# Autodesk Inventor assembly: SPE0V1 Ensamble General
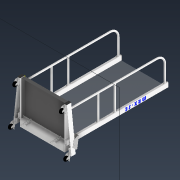
[picture p0: Inventor's stored thumbnail of the model, 180x180]
Saved by Autodesk Inventor 2021.2 (Build 252289000, 289)
## iProperties
Created: 2026-05-12
Part Number: SPE0V1 Ensamble General
Document SubType Name: Assembly
Designer: nelso
Author: nelso
## Documents named in this file (11)
- C:\Users\Tecnica\OneDrive\Documentos\Mecanica\Soporte-Paciente-Espinografia\Workspace\SPE0V1 Ensamble General.iam
- C:\Users\Tecnica\OneDrive\Documentos\Mecanica\Soporte-Paciente-Espinografia\Workspace\SP25V1 Acrilico.ipt
- C:\Users\Tecnica\OneDrive\Documentos\Mecanica\Soporte-Paciente-Espinografia\Workspace\SPE1V1 Estructura.iam
- C:\Users\Tecnica\OneDrive\Documentos\Mecanica\Soporte-Paciente-Espinografia\Workspace\SPE2V1 Baranda.iam
- C:\Users\Tecnica\OneDrive\Documentos\Mecanica\Soporte-Paciente-Espinografia\Workspace\DIN933M8X1.25L20C.ipt
- C:\Users\Tecnica\OneDrive\Documentos\Mecanica\Soporte-Paciente-Espinografia\Workspace\DIN125-A8,4C.ipt
- C:\Users\Tecnica\OneDrive\Documentos\Mecanica\Soporte-Paciente-Espinografia\Workspace\Logo.ipt
- C:\Users\Tecnica\OneDrive\Documentos\Mecanica\Soporte-Paciente-Espinografia\Workspace\SP16V1 Seguro Acrilico.ipt
- C:\Users\Tecnica\OneDrive\Documentos\Mecanica\Soporte-Paciente-Espinografia\Workspace\RFPLUS4PO300 Tuerca rem M4 cab red.ipt
- C:\Users\Tecnica\OneDrive\Documentos\Mecanica\Soporte-Paciente-Espinografia\Workspace\ISO7380M4X0.8L12I.ipt
- C:\Users\Tecnica\OneDrive\Documentos\Mecanica\Soporte-Paciente-Espinografia\Workspace\SP26V1 Base Chapa.ipt
## Components (76 placed, 10 different names)
1. SP26V1 Base Chapa:1 — Flush:17, Mate:178, Mate:242
2. SP25V1 Acrilico:1 — Mate:71, Mate:179, Mate:180, Flush:19, Flush:20, Mate:261, Mate:262
3. SPE1V1 Estructura:1 [sub-assembly] — Mate:71, Coincidencia:100, Coincidencia:101, Coincidencia:102, Coincidencia:117, Nivelación:14, Nivelación:15, Flush:17, Mate:178, Flush:23, Flush:24, Flush:25, Flush:26, Flush:27, Flush:28, Flush:29, Flush:30, Flush:31, Mate:235, Mate:236, Mate:237, Flush:32, Flush:33, Flush:34, Flush:35, Flush:36, Flush:37, Flush:38, Flush:39, Flush:40, Mate:239, Mate:240, Mate:241, Mate:242, Flush:41, Flush:42, Mate:243, Mate:244, Mate:245, Mate:246, Mate:247, Mate:248, Mate:249, Mate:250, Mate:251, Mate:252, Mate:253, Mate:254, Mate:255, Mate:256, Mate:257, Mate:258, Mate:259, Mate:260
4. SPE2V1 Baranda:2 [sub-assembly] — Coincidencia:100, Coincidencia:101, Coincidencia:102, Coincidencia:109, Coincidencia:110, Coincidencia:111, Coincidencia:112, Mate:134, Mate:135, Mate:136, Mate:137, Mate:138, Mate:139, Mate:140, Mate:141, Mate:142, Mate:143, Mate:144, Mate:145, Mate:168, Mate:169, Mate:170, Mate:171, Mate:172, Mate:173
5. SPE2V1 Baranda:3 [sub-assembly] — Mate:118, Mate:119, Mate:120, Mate:121, Mate:122, Mate:123, Mate:124, Mate:125, Mate:126, Mate:127, Mate:128, Mate:129, Mate:130, Mate:131, Mate:132, Mate:133, Mate:147, Mate:149, Mate:156, Mate:157, Mate:158, Mate:159, Mate:160, Mate:161, Mate:235, Mate:236
6. DIN933M8X1.25L20C:1 — Coincidencia:113, Coincidencia:114
7. DIN125-A8,4C:1 — Coincidencia:109, Coincidencia:110, Coincidencia:115, Coincidencia:116
8. DIN125-A8,4C:2 — Coincidencia:111, Coincidencia:112, Coincidencia:113, Coincidencia:114
9. DIN933M8X1.25L20C:2 — Coincidencia:115, Coincidencia:116
10. Logo:1 — Coincidencia:117, Nivelación:14, Nivelación:15
11. DIN125-A8,4C:3 — Mate:144, Mate:145, Mate:162
12. DIN125-A8,4C:4 — Mate:142, Mate:143, Mate:163
13. DIN125-A8,4C:5 — Mate:140, Mate:141, Mate:164
14. DIN125-A8,4C:6 — Mate:138, Mate:139, Mate:165
15. DIN125-A8,4C:7 — Mate:135, Mate:136, Mate:167
16. DIN125-A8,4C:8 — Mate:134, Mate:137, Mate:166
17. DIN125-A8,4C:9 — Mate:130, Mate:132, Mate:155
18. DIN125-A8,4C:10 — Mate:131, Mate:133, Mate:154
19. DIN125-A8,4C:11 — Mate:128, Mate:129, Mate:153
20. DIN125-A8,4C:12 — Mate:126, Mate:127, Mate:152
21. DIN125-A8,4C:13 — Mate:122, Mate:123, Mate:150
22. DIN125-A8,4C:14 — Mate:124, Mate:125, Mate:151
23. DIN125-A8,4C:15 — Mate:120, Mate:121, Mate:148
24. DIN125-A8,4C:16 — Mate:118, Mate:119, Mate:146
25. DIN933M8X1.25L20C:3 — Mate:162, Mate:168
26. DIN933M8X1.25L20C:4 — Mate:163, Mate:169
27. DIN933M8X1.25L20C:5 — Mate:164, Mate:170
28. DIN933M8X1.25L20C:6 — Mate:165, Mate:171
29. DIN933M8X1.25L20C:7 — Mate:166, Mate:172
30. DIN933M8X1.25L20C:8 — Mate:167, Mate:173
31. DIN933M8X1.25L20C:9 — Mate:155, Mate:156
32. DIN933M8X1.25L20C:10 — Mate:154, Mate:157
33. DIN933M8X1.25L20C:11 — Mate:153, Mate:159
34. DIN933M8X1.25L20C:12 — Mate:152, Mate:158
35. DIN933M8X1.25L20C:13 — Mate:151, Mate:160
36. DIN933M8X1.25L20C:14 — Mate:150, Mate:161, Mate:237
37. DIN933M8X1.25L20C:15 — Mate:148, Mate:149
38. DIN933M8X1.25L20C:16 — Mate:146, Mate:147
39. SP16V1 Seguro Acrilico:1 — Mate:179, Flush:19, Mate:181, Mate:199, Mate:200, Mate:201, Mate:202, Mate:203, Mate:204, Mate:205, Mate:206, Mate:207, Mate:217, Mate:218, Mate:219, Mate:220, Mate:221, Mate:222, Mate:223, Mate:224, Mate:225
40. SP16V1 Seguro Acrilico:2 — Mate:180, Flush:20, Mate:208, Mate:209, Mate:210, Mate:211, Mate:212, Mate:213, Mate:214, Mate:215, Mate:216, Mate:226, Mate:227, Mate:228, Mate:229, Mate:230, Mate:231, Mate:232, Mate:233, Mate:234, Flush:40, Flush:42
41. RFPLUS4PO300 Tuerca rem M4 cab red:1 — Mate:181, Flush:23, Mate:251
42. RFPLUS4PO300 Tuerca rem M4 cab red:2 — Flush:24, Mate:250
43. RFPLUS4PO300 Tuerca rem M4 cab red:3 — Flush:25, Mate:249
44. RFPLUS4PO300 Tuerca rem M4 cab red:4 — Flush:26, Mate:248
45. RFPLUS4PO300 Tuerca rem M4 cab red:5 — Flush:27, Mate:247
46. RFPLUS4PO300 Tuerca rem M4 cab red:6 — Flush:28, Mate:246
47. RFPLUS4PO300 Tuerca rem M4 cab red:7 — Flush:29, Mate:245
48. RFPLUS4PO300 Tuerca rem M4 cab red:8 — Flush:30, Mate:244
49. RFPLUS4PO300 Tuerca rem M4 cab red:9 — Flush:31, Mate:243
50. RFPLUS4PO300 Tuerca rem M4 cab red:10 — Flush:32, Mate:252, Mate:261
51. RFPLUS4PO300 Tuerca rem M4 cab red:11 — Flush:33, Mate:253
52. RFPLUS4PO300 Tuerca rem M4 cab red:12 — Flush:34, Mate:254
53. RFPLUS4PO300 Tuerca rem M4 cab red:13 — Flush:35, Mate:255
54. RFPLUS4PO300 Tuerca rem M4 cab red:14 — Flush:36, Mate:256
55. RFPLUS4PO300 Tuerca rem M4 cab red:15 — Flush:37, Mate:257
56. RFPLUS4PO300 Tuerca rem M4 cab red:16 — Flush:38, Mate:258
57. RFPLUS4PO300 Tuerca rem M4 cab red:17 — Flush:39, Mate:259
58. RFPLUS4PO300 Tuerca rem M4 cab red:18 — Flush:41, Mate:260
59. ISO7380M4X0.8L12I:1 — Mate:199, Mate:217
60. ISO7380M4X0.8L12I:2 — Mate:200, Mate:218
61. ISO7380M4X0.8L12I:3 — Mate:201, Mate:219
62. ISO7380M4X0.8L12I:4 — Mate:202, Mate:220
63. ISO7380M4X0.8L12I:5 — Mate:203, Mate:221
64. ISO7380M4X0.8L12I:6 — Mate:204, Mate:222
65. ISO7380M4X0.8L12I:7 — Mate:205, Mate:223
66. ISO7380M4X0.8L12I:8 — Mate:206, Mate:224
67. ISO7380M4X0.8L12I:9 — Mate:207, Mate:225
68. ISO7380M4X0.8L12I:10 — Mate:208, Mate:234, Mate:262
69. ISO7380M4X0.8L12I:11 — Mate:209, Mate:233
70. ISO7380M4X0.8L12I:12 — Mate:210, Mate:232
71. ISO7380M4X0.8L12I:13 — Mate:211, Mate:231
72. ISO7380M4X0.8L12I:14 — Mate:212, Mate:230
73. ISO7380M4X0.8L12I:15 — Mate:214, Mate:228
74. ISO7380M4X0.8L12I:16 — Mate:215, Mate:227
75. ISO7380M4X0.8L12I:17 — Mate:216, Mate:226
76. ISO7380M4X0.8L12I:18 — Mate:213, Mate:229
## Relationships (161: Mate 136, Flush 25)
- Mate:71: SP25V1 Acrilico:1 ↔ SPE1V1 Estructura:1
- Coincidencia:100 [Mate]: SPE1V1 Estructura:1 ↔ SPE2V1 Baranda:2
- Coincidencia:101 [Mate]: SPE1V1 Estructura:1 ↔ SPE2V1 Baranda:2
- Coincidencia:102 [Mate]: SPE1V1 Estructura:1 ↔ SPE2V1 Baranda:2
- Coincidencia:109 [Mate]: SPE2V1 Baranda:2 ↔ DIN125-A8,4C:1
- Coincidencia:110 [Mate]: SPE2V1 Baranda:2 ↔ DIN125-A8,4C:1
- Coincidencia:111 [Mate]: SPE2V1 Baranda:2 ↔ DIN125-A8,4C:2
- Coincidencia:112 [Mate]: SPE2V1 Baranda:2 ↔ DIN125-A8,4C:2
- Coincidencia:113 [Mate]: DIN933M8X1.25L20C:1 ↔ DIN125-A8,4C:2
- Coincidencia:114 [Mate]: DIN933M8X1.25L20C:1 ↔ DIN125-A8,4C:2
- Coincidencia:115 [Mate]: DIN125-A8,4C:1 ↔ DIN933M8X1.25L20C:2
- Coincidencia:116 [Mate]: DIN125-A8,4C:1 ↔ DIN933M8X1.25L20C:2
- Coincidencia:117 [Mate]: SPE1V1 Estructura:1 ↔ Logo:1
- Nivelación:14 [Flush] (10 mm): SPE1V1 Estructura:1 ↔ Logo:1
- Nivelación:15 [Flush] (400 mm): SPE1V1 Estructura:1 ↔ Logo:1
- Mate:118: SPE2V1 Baranda:3 ↔ DIN125-A8,4C:16
- Mate:119: SPE2V1 Baranda:3 ↔ DIN125-A8,4C:16
- Mate:120: SPE2V1 Baranda:3 ↔ DIN125-A8,4C:15
- Mate:121: SPE2V1 Baranda:3 ↔ DIN125-A8,4C:15
- Mate:122: SPE2V1 Baranda:3 ↔ DIN125-A8,4C:13
- Mate:123: SPE2V1 Baranda:3 ↔ DIN125-A8,4C:13
- Mate:124: SPE2V1 Baranda:3 ↔ DIN125-A8,4C:14
- Mate:125: SPE2V1 Baranda:3 ↔ DIN125-A8,4C:14
- Mate:126: SPE2V1 Baranda:3 ↔ DIN125-A8,4C:12
- Mate:127: SPE2V1 Baranda:3 ↔ DIN125-A8,4C:12
- Mate:128: SPE2V1 Baranda:3 ↔ DIN125-A8,4C:11
- Mate:129: SPE2V1 Baranda:3 ↔ DIN125-A8,4C:11
- Mate:130: SPE2V1 Baranda:3 ↔ DIN125-A8,4C:9
- Mate:131: SPE2V1 Baranda:3 ↔ DIN125-A8,4C:10
- Mate:132: SPE2V1 Baranda:3 ↔ DIN125-A8,4C:9
- Mate:133: SPE2V1 Baranda:3 ↔ DIN125-A8,4C:10
- Mate:134: SPE2V1 Baranda:2 ↔ DIN125-A8,4C:8
- Mate:135: SPE2V1 Baranda:2 ↔ DIN125-A8,4C:7
- Mate:136: SPE2V1 Baranda:2 ↔ DIN125-A8,4C:7
- Mate:137: SPE2V1 Baranda:2 ↔ DIN125-A8,4C:8
- Mate:138: SPE2V1 Baranda:2 ↔ DIN125-A8,4C:6
- Mate:139: SPE2V1 Baranda:2 ↔ DIN125-A8,4C:6
- Mate:140: SPE2V1 Baranda:2 ↔ DIN125-A8,4C:5
- Mate:141: SPE2V1 Baranda:2 ↔ DIN125-A8,4C:5
- Mate:142: SPE2V1 Baranda:2 ↔ DIN125-A8,4C:4
- Mate:143: SPE2V1 Baranda:2 ↔ DIN125-A8,4C:4
- Mate:144: SPE2V1 Baranda:2 ↔ DIN125-A8,4C:3
- Mate:145: SPE2V1 Baranda:2 ↔ DIN125-A8,4C:3
- Mate:146: DIN125-A8,4C:16 ↔ DIN933M8X1.25L20C:16
- Mate:147: SPE2V1 Baranda:3 ↔ DIN933M8X1.25L20C:16
- Mate:148: DIN125-A8,4C:15 ↔ DIN933M8X1.25L20C:15
- Mate:149: SPE2V1 Baranda:3 ↔ DIN933M8X1.25L20C:15
- Mate:150: DIN125-A8,4C:13 ↔ DIN933M8X1.25L20C:14
- Mate:151: DIN125-A8,4C:14 ↔ DIN933M8X1.25L20C:13
- Mate:152: DIN125-A8,4C:12 ↔ DIN933M8X1.25L20C:12
- Mate:153: DIN125-A8,4C:11 ↔ DIN933M8X1.25L20C:11
- Mate:154: DIN125-A8,4C:10 ↔ DIN933M8X1.25L20C:10
- Mate:155: DIN125-A8,4C:9 ↔ DIN933M8X1.25L20C:9
- Mate:156: SPE2V1 Baranda:3 ↔ DIN933M8X1.25L20C:9
- Mate:157: SPE2V1 Baranda:3 ↔ DIN933M8X1.25L20C:10
- Mate:158: SPE2V1 Baranda:3 ↔ DIN933M8X1.25L20C:12
- Mate:159: SPE2V1 Baranda:3 ↔ DIN933M8X1.25L20C:11
- Mate:160: SPE2V1 Baranda:3 ↔ DIN933M8X1.25L20C:13
- Mate:161: SPE2V1 Baranda:3 ↔ DIN933M8X1.25L20C:14
- Mate:162: DIN125-A8,4C:3 ↔ DIN933M8X1.25L20C:3
- Mate:163: DIN125-A8,4C:4 ↔ DIN933M8X1.25L20C:4
- Mate:164: DIN125-A8,4C:5 ↔ DIN933M8X1.25L20C:5
- Mate:165: DIN125-A8,4C:6 ↔ DIN933M8X1.25L20C:6
- Mate:166: DIN125-A8,4C:8 ↔ DIN933M8X1.25L20C:7
- Mate:167: DIN125-A8,4C:7 ↔ DIN933M8X1.25L20C:8
- Mate:168: SPE2V1 Baranda:2 ↔ DIN933M8X1.25L20C:3
- Mate:169: SPE2V1 Baranda:2 ↔ DIN933M8X1.25L20C:4
- Mate:170: SPE2V1 Baranda:2 ↔ DIN933M8X1.25L20C:5
- Mate:171: SPE2V1 Baranda:2 ↔ DIN933M8X1.25L20C:6
- Mate:172: SPE2V1 Baranda:2 ↔ DIN933M8X1.25L20C:7
- Mate:173: SPE2V1 Baranda:2 ↔ DIN933M8X1.25L20C:8
- Flush:17: SP26V1 Base Chapa:1 ↔ SPE1V1 Estructura:1
- Mate:178 (5 mm): SP26V1 Base Chapa:1 ↔ SPE1V1 Estructura:1
- Mate:179: SP25V1 Acrilico:1 ↔ SP16V1 Seguro Acrilico:1
- Mate:180: SP25V1 Acrilico:1 ↔ SP16V1 Seguro Acrilico:2
- Flush:19: SP25V1 Acrilico:1 ↔ SP16V1 Seguro Acrilico:1
- Flush:20: SP25V1 Acrilico:1 ↔ SP16V1 Seguro Acrilico:2
- Mate:181: SP16V1 Seguro Acrilico:1 ↔ RFPLUS4PO300 Tuerca rem M4 cab red:1
- Flush:23: SPE1V1 Estructura:1 ↔ RFPLUS4PO300 Tuerca rem M4 cab red:1
- Flush:24: SPE1V1 Estructura:1 ↔ RFPLUS4PO300 Tuerca rem M4 cab red:2
- Flush:25: SPE1V1 Estructura:1 ↔ RFPLUS4PO300 Tuerca rem M4 cab red:3
- Flush:26: SPE1V1 Estructura:1 ↔ RFPLUS4PO300 Tuerca rem M4 cab red:4
- Flush:27: SPE1V1 Estructura:1 ↔ RFPLUS4PO300 Tuerca rem M4 cab red:5
- Flush:28: SPE1V1 Estructura:1 ↔ RFPLUS4PO300 Tuerca rem M4 cab red:6
- Flush:29: SPE1V1 Estructura:1 ↔ RFPLUS4PO300 Tuerca rem M4 cab red:7
- Flush:30: SPE1V1 Estructura:1 ↔ RFPLUS4PO300 Tuerca rem M4 cab red:8
- Flush:31: SPE1V1 Estructura:1 ↔ RFPLUS4PO300 Tuerca rem M4 cab red:9
- Mate:199: SP16V1 Seguro Acrilico:1 ↔ ISO7380M4X0.8L12I:1
- Mate:200: SP16V1 Seguro Acrilico:1 ↔ ISO7380M4X0.8L12I:2
- Mate:201: SP16V1 Seguro Acrilico:1 ↔ ISO7380M4X0.8L12I:3
- Mate:202: SP16V1 Seguro Acrilico:1 ↔ ISO7380M4X0.8L12I:4
- Mate:203: SP16V1 Seguro Acrilico:1 ↔ ISO7380M4X0.8L12I:5
- Mate:204: SP16V1 Seguro Acrilico:1 ↔ ISO7380M4X0.8L12I:6
- Mate:205: SP16V1 Seguro Acrilico:1 ↔ ISO7380M4X0.8L12I:7
- Mate:206: SP16V1 Seguro Acrilico:1 ↔ ISO7380M4X0.8L12I:8
- Mate:207: SP16V1 Seguro Acrilico:1 ↔ ISO7380M4X0.8L12I:9
- Mate:208: SP16V1 Seguro Acrilico:2 ↔ ISO7380M4X0.8L12I:10
- Mate:209: SP16V1 Seguro Acrilico:2 ↔ ISO7380M4X0.8L12I:11
- Mate:210: SP16V1 Seguro Acrilico:2 ↔ ISO7380M4X0.8L12I:12
- Mate:211: SP16V1 Seguro Acrilico:2 ↔ ISO7380M4X0.8L12I:13
- Mate:212: SP16V1 Seguro Acrilico:2 ↔ ISO7380M4X0.8L12I:14
- Mate:213: SP16V1 Seguro Acrilico:2 ↔ ISO7380M4X0.8L12I:18
- Mate:214: SP16V1 Seguro Acrilico:2 ↔ ISO7380M4X0.8L12I:15
- Mate:215: SP16V1 Seguro Acrilico:2 ↔ ISO7380M4X0.8L12I:16
- Mate:216: SP16V1 Seguro Acrilico:2 ↔ ISO7380M4X0.8L12I:17
- Mate:217: SP16V1 Seguro Acrilico:1 ↔ ISO7380M4X0.8L12I:1
- Mate:218: SP16V1 Seguro Acrilico:1 ↔ ISO7380M4X0.8L12I:2
- Mate:219: SP16V1 Seguro Acrilico:1 ↔ ISO7380M4X0.8L12I:3
- Mate:220: SP16V1 Seguro Acrilico:1 ↔ ISO7380M4X0.8L12I:4
- Mate:221: SP16V1 Seguro Acrilico:1 ↔ ISO7380M4X0.8L12I:5
- Mate:222: SP16V1 Seguro Acrilico:1 ↔ ISO7380M4X0.8L12I:6
- Mate:223: SP16V1 Seguro Acrilico:1 ↔ ISO7380M4X0.8L12I:7
- Mate:224: SP16V1 Seguro Acrilico:1 ↔ ISO7380M4X0.8L12I:8
- Mate:225: SP16V1 Seguro Acrilico:1 ↔ ISO7380M4X0.8L12I:9
- Mate:226: SP16V1 Seguro Acrilico:2 ↔ ISO7380M4X0.8L12I:17
- Mate:227: SP16V1 Seguro Acrilico:2 ↔ ISO7380M4X0.8L12I:16
- Mate:228: SP16V1 Seguro Acrilico:2 ↔ ISO7380M4X0.8L12I:15
- Mate:229: SP16V1 Seguro Acrilico:2 ↔ ISO7380M4X0.8L12I:18
- Mate:230: SP16V1 Seguro Acrilico:2 ↔ ISO7380M4X0.8L12I:14
- Mate:231: SP16V1 Seguro Acrilico:2 ↔ ISO7380M4X0.8L12I:13
- Mate:232: SP16V1 Seguro Acrilico:2 ↔ ISO7380M4X0.8L12I:12
- Mate:233: SP16V1 Seguro Acrilico:2 ↔ ISO7380M4X0.8L12I:11
- Mate:234: SP16V1 Seguro Acrilico:2 ↔ ISO7380M4X0.8L12I:10
- Mate:235: SPE1V1 Estructura:1 ↔ SPE2V1 Baranda:3
- Mate:236: SPE1V1 Estructura:1 ↔ SPE2V1 Baranda:3
- Mate:237: SPE1V1 Estructura:1 ↔ DIN933M8X1.25L20C:14
- Flush:32: SPE1V1 Estructura:1 ↔ RFPLUS4PO300 Tuerca rem M4 cab red:10
- Flush:33: SPE1V1 Estructura:1 ↔ RFPLUS4PO300 Tuerca rem M4 cab red:11
- Flush:34: SPE1V1 Estructura:1 ↔ RFPLUS4PO300 Tuerca rem M4 cab red:12
- Flush:35: SPE1V1 Estructura:1 ↔ RFPLUS4PO300 Tuerca rem M4 cab red:13
- Flush:36: SPE1V1 Estructura:1 ↔ RFPLUS4PO300 Tuerca rem M4 cab red:14
- Flush:37: SPE1V1 Estructura:1 ↔ RFPLUS4PO300 Tuerca rem M4 cab red:15
- Flush:38: SPE1V1 Estructura:1 ↔ RFPLUS4PO300 Tuerca rem M4 cab red:16
- Flush:39: SPE1V1 Estructura:1 ↔ RFPLUS4PO300 Tuerca rem M4 cab red:17
- Flush:40: SPE1V1 Estructura:1 ↔ SP16V1 Seguro Acrilico:2
- Mate:239: SPE1V1 Estructura:1
- Mate:240: SPE1V1 Estructura:1
- Mate:241: SPE1V1 Estructura:1
- Mate:242: SP26V1 Base Chapa:1 ↔ SPE1V1 Estructura:1
- Flush:41: SPE1V1 Estructura:1 ↔ RFPLUS4PO300 Tuerca rem M4 cab red:18
- Flush:42: SPE1V1 Estructura:1 ↔ SP16V1 Seguro Acrilico:2
- Mate:243: SPE1V1 Estructura:1 ↔ RFPLUS4PO300 Tuerca rem M4 cab red:9
- Mate:244: SPE1V1 Estructura:1 ↔ RFPLUS4PO300 Tuerca rem M4 cab red:8
- Mate:245: SPE1V1 Estructura:1 ↔ RFPLUS4PO300 Tuerca rem M4 cab red:7
- Mate:246: SPE1V1 Estructura:1 ↔ RFPLUS4PO300 Tuerca rem M4 cab red:6
- Mate:247: SPE1V1 Estructura:1 ↔ RFPLUS4PO300 Tuerca rem M4 cab red:5
- Mate:248: SPE1V1 Estructura:1 ↔ RFPLUS4PO300 Tuerca rem M4 cab red:4
- Mate:249: SPE1V1 Estructura:1 ↔ RFPLUS4PO300 Tuerca rem M4 cab red:3
- Mate:250: SPE1V1 Estructura:1 ↔ RFPLUS4PO300 Tuerca rem M4 cab red:2
- Mate:251: SPE1V1 Estructura:1 ↔ RFPLUS4PO300 Tuerca rem M4 cab red:1
- Mate:252: SPE1V1 Estructura:1 ↔ RFPLUS4PO300 Tuerca rem M4 cab red:10
- Mate:253: SPE1V1 Estructura:1 ↔ RFPLUS4PO300 Tuerca rem M4 cab red:11
- Mate:254: SPE1V1 Estructura:1 ↔ RFPLUS4PO300 Tuerca rem M4 cab red:12
- Mate:255: SPE1V1 Estructura:1 ↔ RFPLUS4PO300 Tuerca rem M4 cab red:13
- Mate:256: SPE1V1 Estructura:1 ↔ RFPLUS4PO300 Tuerca rem M4 cab red:14
- Mate:257: SPE1V1 Estructura:1 ↔ RFPLUS4PO300 Tuerca rem M4 cab red:15
- Mate:258: SPE1V1 Estructura:1 ↔ RFPLUS4PO300 Tuerca rem M4 cab red:16
- Mate:259: SPE1V1 Estructura:1 ↔ RFPLUS4PO300 Tuerca rem M4 cab red:17
- Mate:260: SPE1V1 Estructura:1 ↔ RFPLUS4PO300 Tuerca rem M4 cab red:18
- Mate:261: SP25V1 Acrilico:1 ↔ RFPLUS4PO300 Tuerca rem M4 cab red:10
- Mate:262: SP25V1 Acrilico:1 ↔ ISO7380M4X0.8L12I:10
